# Autodesk Inventor assembly: 齿轮箱1
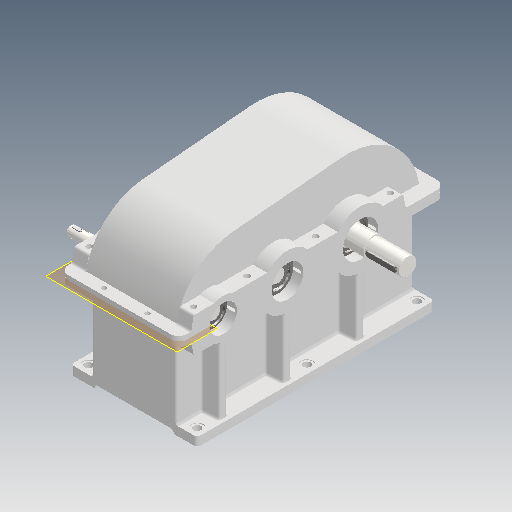
[picture p0: Inventor's stored thumbnail of the model, 512x512]
Saved by Autodesk Inventor 2025 (Build 290162000, 162)
## iProperties
Created: 2025-03-10
Part Number: 齿轮箱1
Document SubType Name: Assembly
Designer: liukan
Author: liukan
## Documents named in this file (12)
- E:\Autodesk\Inventor files\齿轮箱1.iam
- E:\Autodesk\Inventor files\下半箱体.ipt
- E:\Autodesk\Inventor files\高速轴.iam
- E:\Autodesk\Inventor files\中间轴.iam
- E:\Autodesk\Inventor files\低速轴.iam
- E:\Autodesk\Inventor files\高速齿轮.iam
- E:\Autodesk\Inventor files\低速齿轮.iam
- E:\Autodesk\Inventor files\齿轮箱1\设计加速器\键联接1.iam
- E:\Autodesk\Inventor files\齿轮箱1\设计加速器\键联接2.iam
- E:\Autodesk\Inventor files\齿轮箱1\设计加速器\键联接3.iam
- E:\Autodesk\Inventor files\齿轮箱1\设计加速器\键联接4.iam
- E:\Autodesk\Inventor files\上半箱体.ipt
## Components (11 placed, 8 different names)
1. 下半箱体:1 — 表面齐平:1, 表面齐平:2, 表面齐平:3, 角度:1, 表面齐平:4, 配合:15, 表面齐平:12, 表面齐平:13
2. 上半箱体:1 — 表面齐平:12, 表面齐平:13
3. 高速轴:1 [sub-assembly] — 角度:1, 配合:2, 表面齐平:9, 表面齐平:11
4. 中间轴:1 [sub-assembly] — 角度:2, 配合:1, 配合:5, 配合:6, 角度:9, 配合:8, 表面齐平:6, 角度:10, 配合:9, 角度:11, 表面齐平:7, 角度:12, 配合:10, 配合:13, 表面齐平:9, 配合:15
5. 低速轴:1 [sub-assembly] — 角度:3, 配合:4, 角度:7, 表面齐平:4, 配合:6, 表面齐平:8, 角度:13, 配合:11, 角度:14, 配合:12, 配合:13, 表面齐平:10, 角度:15, 配合:14
6. 高速齿轮:1 [sub-assembly] — 配合:1, 配合:2, 角度:4, 角度:9, 配合:8
7. 低速齿轮:1 [sub-assembly] — 配合:4, 配合:5, 角度:11, 角度:14, 配合:12
8. 键联接:1 [sub-assembly] — 表面齐平:7, 角度:12, 配合:10
9. 键联接:2 [sub-assembly] — 表面齐平:6, 角度:10, 配合:9
10. 键联接:3 [sub-assembly] — 表面齐平:8, 角度:13, 配合:11
11. 键联接:4 [sub-assembly] — 表面齐平:10, 角度:15, 配合:14
## Relationships (37: Mate 13, Flush 12, Angle 12)
- 表面齐平:1 [Flush]: 下半箱体:1
- 表面齐平:2 [Flush]: 下半箱体:1
- 表面齐平:3 [Flush]: 下半箱体:1
- 角度:1 [Angle] (0 deg): 下半箱体:1 ↔ 高速轴:1
- 角度:2 [Angle] (0 deg): 中间轴:1
- 角度:3 [Angle] (0 deg): 低速轴:1
- 配合:1 [Mate]: 中间轴:1 ↔ 高速齿轮:1
- 配合:2 [Mate]: 高速轴:1 ↔ 高速齿轮:1
- 角度:4 [Angle] (180 deg): 高速齿轮:1
- 配合:4 [Mate]: 低速轴:1 ↔ 低速齿轮:1
- 配合:5 [Mate]: 中间轴:1 ↔ 低速齿轮:1
- 角度:7 [Angle] (0 deg): 低速轴:1
- 表面齐平:4 [Flush]: 下半箱体:1 ↔ 低速轴:1
- 配合:6 [Mate]: 中间轴:1 ↔ 低速轴:1
- 角度:9 [Angle] (11.4804 deg): 中间轴:1 ↔ 高速齿轮:1
- 配合:8 [Mate]: 中间轴:1 ↔ 高速齿轮:1
- 表面齐平:6 [Flush] (10 mm): 中间轴:1 ↔ 键联接:2
- 角度:10 [Angle] (0 deg): 中间轴:1 ↔ 键联接:2
- 配合:9 [Mate]: 中间轴:1 ↔ 键联接:2
- 角度:11 [Angle] (170.0196 deg): 中间轴:1 ↔ 低速齿轮:1
- 表面齐平:7 [Flush] (8 mm): 中间轴:1 ↔ 键联接:1
- 角度:12 [Angle] (0 deg): 中间轴:1 ↔ 键联接:1
- 配合:10 [Mate]: 中间轴:1 ↔ 键联接:1
- 表面齐平:8 [Flush] (6 mm): 低速轴:1 ↔ 键联接:3
- 角度:13 [Angle] (0 deg): 低速轴:1 ↔ 键联接:3
- 配合:11 [Mate]: 低速轴:1 ↔ 键联接:3
- 角度:14 [Angle] (88.2353 deg): 低速轴:1 ↔ 低速齿轮:1
- 配合:12 [Mate]: 低速轴:1 ↔ 低速齿轮:1
- 配合:13 [Mate]: 中间轴:1 ↔ 低速轴:1
- 表面齐平:9 [Flush]: 高速轴:1 ↔ 中间轴:1
- 表面齐平:10 [Flush] (5 mm): 低速轴:1 ↔ 键联接:4
- 角度:15 [Angle] (0 deg): 低速轴:1 ↔ 键联接:4
- 配合:14 [Mate]: 低速轴:1 ↔ 键联接:4
- 表面齐平:11 [Flush] (289 mm): 高速轴:1
- 配合:15 [Mate]: 下半箱体:1 ↔ 中间轴:1
- 表面齐平:12 [Flush]: 下半箱体:1 ↔ 上半箱体:1
- 表面齐平:13 [Flush]: 下半箱体:1 ↔ 上半箱体:1
